# Autodesk Inventor assembly: FinalAssembly
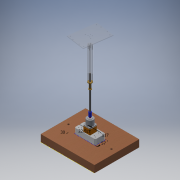
[picture p0: Inventor's stored thumbnail of the model, 180x180]
Saved by Autodesk Inventor 2019 (Build 230136000, 136)
## iProperties
Created: 2019-05-17
Part Number: FinalAssembly
Document SubType Name: Assembly
Designer: Iván
Author: Iván
## Documents named in this file (9)
- C:\Users\Iván\Documents\Github\RMTestMachine\3DModel\FinalAssembly.iam
- C:\Users\Iván\Documents\Github\RMTestMachine\3DModel\TablaInferior.ipt
- C:\Users\Iván\Documents\Github\RMTestMachine\3DModel\FreeCAD\pieza3.ipt
- C:\Users\Iván\Documents\Github\RMTestMachine\3DModel\motor con reductora.ipt
- C:\Users\Iván\Documents\Github\RMTestMachine\3DModel\AcopleMotor.ipt
- C:\Users\Iván\Documents\Github\RMTestMachine\3DModel\BarraRoscadaT8.ipt
- C:\Users\Iván\Documents\Github\RMTestMachine\3DModel\tuerca anti backlash.ipt
- C:\Users\Iván\Documents\Github\RMTestMachine\3DModel\BarraSolidaMotor.ipt
- C:\Users\Iván\Documents\Github\RMTestMachine\3DModel\base inferior.ipt
## Components (8 placed, 8 different names)
1. TablaInferior:1 — Mate:1, Mate:2, Insert:1, Mate:3, Angle:1
2. pieza3:1 — Insert:1, Angle:1, Mate:4, Mate:5
3. motor con reductora:1 — Mate:4, Mate:5, Insert:2
4. AcopleMotor:1 — Insert:2, Insert:3
5. BarraRoscadaT8:1 — Insert:3, Insert:4
6. tuerca anti backlash:1 — Insert:4, Mate:6, Mate:7
7. BarraSolidaMotor:1 — Mate:6, Mate:7, Insert:5
8. base inferior:1 — Insert:5
## Relationships (13: Mate 7, Insert 5, Angle 1)
- Mate:1: TablaInferior:1
- Mate:2: TablaInferior:1
- Insert:1: TablaInferior:1 ↔ pieza3:1
- Mate:3: TablaInferior:1
- Angle:1 (0 deg): TablaInferior:1 ↔ pieza3:1
- Mate:4: pieza3:1 ↔ motor con reductora:1
- Mate:5: pieza3:1 ↔ motor con reductora:1
- Insert:2 (-12.7 mm): motor con reductora:1 ↔ AcopleMotor:1
- Insert:3 (-12.7 mm): AcopleMotor:1 ↔ BarraRoscadaT8:1
- Insert:4 (-80 mm): BarraRoscadaT8:1 ↔ tuerca anti backlash:1
- Mate:6: tuerca anti backlash:1 ↔ BarraSolidaMotor:1
- Mate:7: tuerca anti backlash:1 ↔ BarraSolidaMotor:1
- Insert:5 (40 mm): BarraSolidaMotor:1 ↔ base inferior:1
